# Autodesk Inventor assembly: 左脚中間ユニット2_MIR
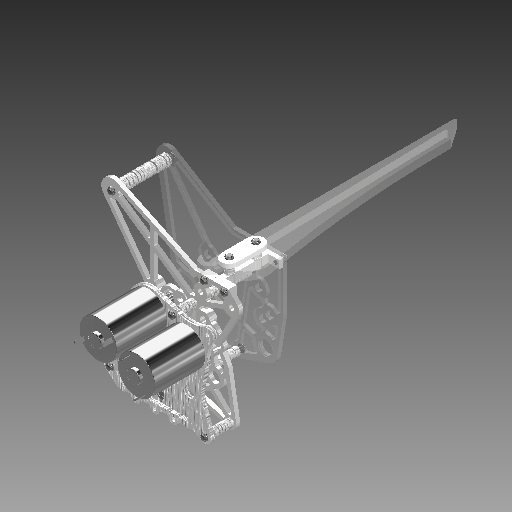
[picture p0: Inventor's stored thumbnail of the model, 512x512]
Saved by Autodesk Inventor 2020 (Build 240168000, 168)
## iProperties
Created: 2019-09-03
Part Number: 左脚中間ユニット2_MIR
Document SubType Name: Assembly
Designer: 雪村
Mass: 302.736 g
Surface Area: 871.212 cm^2
Volume: 107.328 cm^3
Density: 2.82066 g/cm^3
Author: 雪村
## Documents named in this file (23)
- C:\Users\white\Documents\SRDC\SRDC\Inventor_2017\2018年機体\2020年4年機体\右脚中間ユニット2.iam
- C:\Users\white\Documents\SRDC\SRDC\Inventor_2017\2018年機体\2020年4年機体\脚モーターマウントフレーム2_MIR.ipt
- C:\Users\white\Documents\SRDC\SRDC\Inventor_2017\2018年機体\パーツ\RS-380.8.iam
- C:\Users\white\Documents\SRDC\SRDC\Inventor_2017\2018年機体\2020年4年機体\歯車m0.5,z80(樹脂).ipt
- C:\Users\white\Documents\SRDC\SRDC\Inventor_2017\2018年機体\2020年4年機体\歯車m2.z7(z19).ipt
- C:\Users\white\Documents\SRDC\SRDC\Inventor_2017\2018年機体\2020年4年機体\脚中間内フレーム5_MIR.ipt
- C:\Users\white\Documents\SRDC\SRDC\Inventor_2017\2018年機体\2020年4年機体\脚中間跨ぎフレーム1_MIR.ipt
- C:\Users\white\Documents\SRDC\SRDC\Inventor_2017\2018年機体\パーツ\ベアリングフランジ付き040904.ipt
- C:\Users\white\Documents\SRDC\SRDC\Inventor_2017\2018年機体\パーツ\シムリング0406,0.5t.ipt
- C:\Users\white\Documents\SRDC\SRDC\Inventor_2017\2018年機体\パーツ\スペーサーm3,13.ipt
- C:\Users\white\Documents\SRDC\SRDC\Inventor_2017\2018年機体\パーツ\スペーサーm3,16.ipt
- C:\Users\white\Documents\SRDC\SRDC\Inventor_2017\2018年機体\2020年4年機体\脚中間外フレーム3_MIR.ipt
- C:\Users\white\Documents\SRDC\SRDC\Inventor_2017\2018年機体\パーツ\平行ピンΦ4.20.ipt
- C:\Users\white\Documents\SRDC\SRDC\Inventor_2017\2018年機体\パーツ\スペーサーm3,38,Φ8,自作.ipt
- C:\Users\white\Documents\SRDC\SRDC\Inventor_2017\2018年機体\パーツ\ネジ鍋m3,08.ipt
- C:\Users\white\Documents\SRDC\SRDC\Inventor_2017\2018年機体\パーツ\ネジ鍋m3,06.ipt
- C:\Users\white\Documents\SRDC\SRDC\Inventor_2017\2018年機体\パーツ\ネジ鍋m3,25.ipt
- C:\Users\white\Documents\SRDC\SRDC\Inventor_2017\2018年機体\パーツ\ネジ鍋m2.6,06.ipt
- C:\Users\white\Documents\SRDC\SRDC\Inventor_2017\2018年機体\2020年4年機体\ウイング1_MIR.iam
- C:\Users\white\Documents\SRDC\SRDC\Inventor_2017\2018年機体\パーツ\ネジ皿m3,26.ipt
- C:\Users\white\Documents\SRDC\SRDC\Inventor_2017\2018年機体\パーツ\スペーサーm3,38 自作.ipt
- C:\Users\white\Documents\SRDC\SRDC\Inventor_2017\2018年機体\パーツ\スペーサーm3,17.ipt
- C:\Users\white\Documents\SRDC\SRDC\Inventor_2017\2018年機体\パーツ\ネジ鍋m3,30.ipt
## Components (50 placed, 22 different names)
1. 脚モーターマウントフレーム2_MIR:1 — フラッシュ:1, 挿入:13, 挿入:14, 挿入:15, 挿入:16, 挿入:17, 挿入:33, 挿入:34, メイト:1, メイト:2, 挿入:35, 挿入:36, 挿入:38, 挿入:48, 挿入:50, 挿入:51, 挿入:52, 挿入:53, 挿入:58, 挿入:59
2. RS-380.8:1 [sub-assembly] — 挿入:33, メイト:2
3. RS-380.8:2 [sub-assembly] — 挿入:34, メイト:1
4. 歯車m0.5,z80(樹脂):1 — 挿入:4, 挿入:3
5. 歯車m2.z7(z19):1 — 挿入:4, 挿入:3, 挿入:11, 挿入:12
6. 脚中間内フレーム5_MIR:1 — 挿入:23, 挿入:22, 挿入:24, 挿入:37, 挿入:49, 挿入:62, 挿入:67, 挿入:68, 挿入:69, 挿入:70
7. 脚中間跨ぎフレーム1_MIR:1 — 挿入:23, 挿入:22, 挿入:18, 挿入:20, 挿入:19, 挿入:41, 挿入:42, 挿入:45, 挿入:46, 挿入:47, 挿入:63
8. ベアリングフランジ付き040904:1 — 挿入:13, 挿入:8, 挿入:32
9. ベアリングフランジ付き040904:2 — 挿入:10
10. シムリング0406,0.5t:1 — 挿入:11, 挿入:5
11. シムリング0406,0.5t:2 — 挿入:5, 挿入:9
12. シムリング0406,0.5t:3 — 挿入:6, 挿入:7
13. シムリング0406,0.5t:4 — 挿入:9, 挿入:6
14. シムリング0406,0.5t:5 — 挿入:8, 挿入:7
15. シムリング0406,0.5t:6 — 挿入:12, 挿入:10
16. スペーサーm3,13:1 — 挿入:18, 挿入:14
17. スペーサーm3,13:2 — 挿入:20, 挿入:15
18. スペーサーm3,13:3 — 挿入:19, 挿入:16
19. スペーサーm3,16:1 — 挿入:24, 挿入:17
20. 脚中間外フレーム3_MIR:1 — 挿入:33, 挿入:43, 挿入:44, 挿入:56, 挿入:57, 挿入:71, 挿入:72, 挿入:73
21. 平行ピンΦ4.20:1 — 挿入:32
22. スペーサーm3,38,Φ8,自作:1 — 挿入:33, 挿入:63
23. スペーサーm3,16:2 — 挿入:35
24. ネジ鍋m3,08:1 — 挿入:37
25. ネジ鍋m3,08:2 — 挿入:36
26. ネジ鍋m3,06:1 — 挿入:46
27. ネジ鍋m3,06:2 — 挿入:45
28. ネジ鍋m3,06:3 — 挿入:43
29. ネジ鍋m3,06:4 — 挿入:44
30. ネジ鍋m3,08:3 — 挿入:56
31. ネジ鍋m3,08:4 — 挿入:47
32. ネジ鍋m3,08:5 — 挿入:48
33. ネジ鍋m3,08:6 — 挿入:57
34. ネジ鍋m3,08:8 — 挿入:49
35. ネジ鍋m3,25:2 — 挿入:38
36. ネジ鍋m2.6,06:1 — 挿入:52
37. ネジ鍋m2.6,06:2 — 挿入:53
38. ネジ鍋m2.6,06:3 — 挿入:51
39. ネジ鍋m2.6,06:4 — 挿入:50
40. ウイング1_MIR:1 [sub-assembly] — 挿入:41, 挿入:42
41. ネジ皿m3,26:1 — 挿入:58
42. ネジ皿m3,26:2 — 挿入:59
43. スペーサーm3,38 自作:3 — 挿入:62
44. ネジ鍋m3,06:5 — 挿入:67
45. ネジ鍋m3,06:6 — 挿入:68
46. スペーサーm3,38 自作:4 — 挿入:69
47. スペーサーm3,16:4 — 挿入:70
48. スペーサーm3,17:2 — 挿入:71
49. ネジ鍋m3,08:10 — 挿入:73
50. ネジ鍋m3,30:2 — 挿入:72
## Relationships (58: Insert 55, Mate 2, Flush 1)
- フラッシュ:1 [Flush] (-45 mm): 脚モーターマウントフレーム2_MIR:1
- 挿入:4 [Insert]: 歯車m0.5,z80(樹脂):1 ↔ 歯車m2.z7(z19):1
- 挿入:3 [Insert]: 歯車m0.5,z80(樹脂):1 ↔ 歯車m2.z7(z19):1
- 挿入:23 [Insert]: 脚中間内フレーム5_MIR:1 ↔ 脚中間跨ぎフレーム1_MIR:1
- 挿入:22 [Insert]: 脚中間内フレーム5_MIR:1 ↔ 脚中間跨ぎフレーム1_MIR:1
- 挿入:13 [Insert]: 脚モーターマウントフレーム2_MIR:1 ↔ ベアリングフランジ付き040904:1
- 挿入:11 [Insert]: 歯車m2.z7(z19):1 ↔ シムリング0406,0.5t:1
- 挿入:5 [Insert]: シムリング0406,0.5t:1 ↔ シムリング0406,0.5t:2
- 挿入:9 [Insert]: シムリング0406,0.5t:2 ↔ シムリング0406,0.5t:4
- 挿入:6 [Insert]: シムリング0406,0.5t:3 ↔ シムリング0406,0.5t:4
- 挿入:8 [Insert]: ベアリングフランジ付き040904:1 ↔ シムリング0406,0.5t:5
- 挿入:7 [Insert]: シムリング0406,0.5t:3 ↔ シムリング0406,0.5t:5
- 挿入:12 [Insert]: 歯車m2.z7(z19):1 ↔ シムリング0406,0.5t:6
- 挿入:10 [Insert]: ベアリングフランジ付き040904:2 ↔ シムリング0406,0.5t:6
- 挿入:18 [Insert]: 脚中間跨ぎフレーム1_MIR:1 ↔ スペーサーm3,13:1
- 挿入:14 [Insert]: 脚モーターマウントフレーム2_MIR:1 ↔ スペーサーm3,13:1
- 挿入:20 [Insert]: 脚中間跨ぎフレーム1_MIR:1 ↔ スペーサーm3,13:2
- 挿入:15 [Insert]: 脚モーターマウントフレーム2_MIR:1 ↔ スペーサーm3,13:2
- 挿入:19 [Insert]: 脚中間跨ぎフレーム1_MIR:1 ↔ スペーサーm3,13:3
- 挿入:16 [Insert]: 脚モーターマウントフレーム2_MIR:1 ↔ スペーサーm3,13:3
- 挿入:24 [Insert]: 脚中間内フレーム5_MIR:1 ↔ スペーサーm3,16:1
- 挿入:17 [Insert]: 脚モーターマウントフレーム2_MIR:1 ↔ スペーサーm3,16:1
- 挿入:32 [Insert]: ベアリングフランジ付き040904:1 ↔ 平行ピンΦ4.20:1
- 挿入:33 [Insert]: 脚中間外フレーム3_MIR:1 ↔ スペーサーm3,38,Φ8,自作:1
- 挿入:33 [Insert]: 脚モーターマウントフレーム2_MIR:1 ↔ RS-380.8:1
- 挿入:34 [Insert]: 脚モーターマウントフレーム2_MIR:1 ↔ RS-380.8:2
- メイト:1 [Mate]: 脚モーターマウントフレーム2_MIR:1 ↔ RS-380.8:2
- メイト:2 [Mate]: 脚モーターマウントフレーム2_MIR:1 ↔ RS-380.8:1
- 挿入:35 [Insert]: 脚モーターマウントフレーム2_MIR:1 ↔ スペーサーm3,16:2
- 挿入:36 [Insert]: 脚モーターマウントフレーム2_MIR:1 ↔ ネジ鍋m3,08:2
- 挿入:37 [Insert]: 脚中間内フレーム5_MIR:1 ↔ ネジ鍋m3,08:1
- 挿入:38 [Insert]: 脚モーターマウントフレーム2_MIR:1 ↔ ネジ鍋m3,25:2
- 挿入:41 [Insert]: 脚中間跨ぎフレーム1_MIR:1 ↔ ウイング1_MIR:1
- 挿入:42 [Insert]: 脚中間跨ぎフレーム1_MIR:1 ↔ ウイング1_MIR:1
- 挿入:43 [Insert]: 脚中間外フレーム3_MIR:1 ↔ ネジ鍋m3,06:3
- 挿入:44 [Insert]: 脚中間外フレーム3_MIR:1 ↔ ネジ鍋m3,06:4
- 挿入:45 [Insert]: 脚中間跨ぎフレーム1_MIR:1 ↔ ネジ鍋m3,06:2
- 挿入:46 [Insert]: 脚中間跨ぎフレーム1_MIR:1 ↔ ネジ鍋m3,06:1
- 挿入:47 [Insert]: 脚中間跨ぎフレーム1_MIR:1 ↔ ネジ鍋m3,08:4
- 挿入:48 [Insert]: 脚モーターマウントフレーム2_MIR:1 ↔ ネジ鍋m3,08:5
- 挿入:49 [Insert]: 脚中間内フレーム5_MIR:1 ↔ ネジ鍋m3,08:8
- 挿入:50 [Insert]: 脚モーターマウントフレーム2_MIR:1 ↔ ネジ鍋m2.6,06:4
- 挿入:51 [Insert]: 脚モーターマウントフレーム2_MIR:1 ↔ ネジ鍋m2.6,06:3
- 挿入:52 [Insert]: 脚モーターマウントフレーム2_MIR:1 ↔ ネジ鍋m2.6,06:1
- 挿入:53 [Insert]: 脚モーターマウントフレーム2_MIR:1 ↔ ネジ鍋m2.6,06:2
- 挿入:56 [Insert]: 脚中間外フレーム3_MIR:1 ↔ ネジ鍋m3,08:3
- 挿入:57 [Insert]: 脚中間外フレーム3_MIR:1 ↔ ネジ鍋m3,08:6
- 挿入:58 [Insert]: 脚モーターマウントフレーム2_MIR:1 ↔ ネジ皿m3,26:1
- 挿入:59 [Insert]: 脚モーターマウントフレーム2_MIR:1 ↔ ネジ皿m3,26:2
- 挿入:62 [Insert]: 脚中間内フレーム5_MIR:1 ↔ スペーサーm3,38 自作:3
- 挿入:63 [Insert]: 脚中間跨ぎフレーム1_MIR:1 ↔ スペーサーm3,38,Φ8,自作:1
- 挿入:67 [Insert]: 脚中間内フレーム5_MIR:1 ↔ ネジ鍋m3,06:5
- 挿入:68 [Insert]: 脚中間内フレーム5_MIR:1 ↔ ネジ鍋m3,06:6
- 挿入:69 [Insert]: 脚中間内フレーム5_MIR:1 ↔ スペーサーm3,38 自作:4
- 挿入:70 [Insert]: 脚中間内フレーム5_MIR:1 ↔ スペーサーm3,16:4
- 挿入:71 [Insert]: 脚中間外フレーム3_MIR:1 ↔ スペーサーm3,17:2
- 挿入:72 [Insert]: 脚中間外フレーム3_MIR:1 ↔ ネジ鍋m3,30:2
- 挿入:73 [Insert]: 脚中間外フレーム3_MIR:1 ↔ ネジ鍋m3,08:10
